# Autodesk Inventor assembly: Schlitten
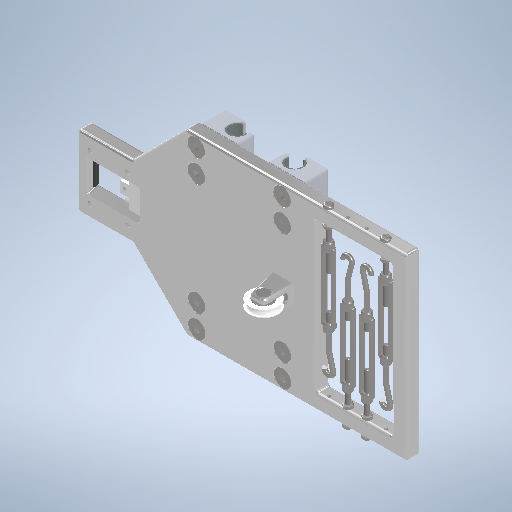
[picture p0: Inventor's stored thumbnail of the model, 512x512]
Saved by Autodesk Inventor 2025 (Build 290162010, 162A)
## iProperties
Created: 2024-11-25
Part Number: Schlitten
Document SubType Name: Assembly
Designer: Admin
Mass: 1140.3 g
Surface Area: 1828.97 cm^2
Volume: 452.563 cm^3
Density: 2.51965 g/cm^3
Author: Admin
## Documents named in this file (25)
- C:\Users\Admin\GIT\HDVKBM\CAD\Krandemonstrator\Schlitten.iam
- C:\Users\Admin\Documents\Inventor\Content Center Files\R2025\de-DE\BS 1804\BS 1804-2 - 2 x 10.ipt
- C:\Users\Admin\GIT\HDVKBM\CAD\Krandemonstrator\SchlittenS.ipt
- C:\Users\Admin\GIT\HDVKBM\CAD\Krandemonstrator\WJ200UM_01_10_1\WJ200UM_01_10_1.iam
- C:\Users\Admin\Documents\Inventor\Content Center Files\R2025\de-DE\DIN 7991(2)\DIN 7991 - M6x16.ipt
- C:\Users\Admin\Documents\Inventor\Content Center Files\R2025\de-DE\AS 1427(03)\AS 1427 - M2 x 10(1).ipt
- C:\Users\Admin\GIT\HDVKBM\CAD\Krandemonstrator\UmlenkrolleHalterHeavy.iam
- C:\Users\Admin\Documents\Inventor\Content Center Files\R2025\de-DE\DIN 7991(2)\DIN 7991 - M3x10.ipt
- C:\Users\Admin\GIT\HDVKBM\CAD\Krandemonstrator\Bremsbelag.ipt
- C:\Users\Admin\GIT\HDVKBM\CAD\Krandemonstrator\BremsePress.ipt
- C:\Users\Admin\GIT\HDVKBM\CAD\Krandemonstrator\Sliderhalterpress.ipt
- C:\Users\Admin\GIT\HDVKBM\CAD\Krandemonstrator\SchubstangeAPress.ipt
- C:\Users\Admin\GIT\HDVKBM\CAD\Krandemonstrator\SchubstangeAPressB.ipt
- C:\Users\Admin\GIT\HDVKBM\CAD\Krandemonstrator\SliderhalterpressB.ipt
- C:\Users\Admin\GIT\HDVKBM\CAD\Krandemonstrator\Druckfeder15.ipt
- C:\Users\Admin\GIT\HDVKBM\CAD\Krandemonstrator\Druckfeder16.ipt
- C:\Users\Admin\Documents\Inventor\Content Center Files\R2025\de-DE\DIN 934\DIN 934 - M3 x 0,5.ipt
- C:\Users\Admin\Documents\Inventor\Content Center Files\R2025\de-DE\AS 1427(01)\AS 1427 - M3 x 40(3).ipt
- C:\Users\Admin\GIT\HDVKBM\CAD\Krandemonstrator\Spannschloss M3-wie din1480.ipt
- C:\Users\Admin\GIT\HDVKBM\CAD\Krandemonstrator\M3 Haken 40mm.ipt
- C:\Users\Admin\Documents\Inventor\Content Center Files\R2025\de-DE\BS EN 28 740\ISO 8740 - 2 x 30(1).ipt
- C:\Users\Admin\GIT\HDVKBM\CAD\Krandemonstrator\Zugfeder16.ipt
- C:\Users\Admin\GIT\HDVKBM\CAD\PrintB\BremsbelagBreit.ipt
- C:\Users\Admin\GIT\HDVKBM\CAD\PrintB\Bauteil8.ipt
- C:\Users\Admin\Documents\Inventor\Content Center Files\R2025\de-DE\AS 1427(01)\AS 1427 - M3 x 35(3).ipt
## Components (57 placed, 23 different names)
1. SchlittenS:1 — Passend:1, Passend:2, Passend:3, Passend:4, Starr:17, Starr:15, Starr:18, Starr:16, Starr:2, Starr:3, Planar:6, Drehbar:9, Zylindrisch:33, Zylindrisch:35, Planar:8, Zylindrisch:39, Passend:40, Passend:41, Passend:42, Passend:43, Zylindrisch:40, Zylindrisch:41, Planar:10, Zylindrisch:50, Zylindrisch:51, Zylindrisch:52, Starr:34, Starr:35, Starr:36, Starr:37, Starr:38, Starr:39, Passend:50, Passend:52, Passend:54, Passend:56, Starr:48, Verschiebbar:34, Verschiebbar:32
2. DIN 7991 M3x10:6 — Zylindrisch:41
3. DIN 7991 M3x10:5 — Zylindrisch:40
4. DIN 934 - ersetzt durch DIN EN 24032/28673/28674 M3:2 — Passend:49, Passend:50
5. DIN 934 - ersetzt durch DIN EN 24032/28673/28674 M3:3 — Passend:51, Passend:52
6. DIN 934 - ersetzt durch DIN EN 24032/28673/28674 M3:4 — Passend:53, Passend:54
7. DIN 934 - ersetzt durch DIN EN 24032/28673/28674 M3:5 — Passend:55, Passend:56
8. AS 1427 - Metrisch M3 x 40:4 — Starr:36, Passend:53, Starr:40
9. AS 1427 - Metrisch M3 x 40:1 — Starr:38, Passend:51, Starr:43
10. AS 1427 - Metrisch M3 x 40:2 — Starr:39, Passend:49, Starr:42
11. AS 1427 - Metrisch M3 x 40:3 — Starr:37, Passend:55, Starr:41
12. Spannschloss M3-wie din1480:1 — Starr:40, Starr:45
13. Spannschloss M3-wie din1480:2 — Starr:41, Starr:44
14. Spannschloss M3-wie din1480:3 — Starr:42, Starr:47
15. Spannschloss M3-wie din1480:4 — Starr:43, Starr:46
16. M3 Haken 40mm:1 — Starr:44
17. M3 Haken 40mm:2 — Starr:45
18. M3 Haken 40mm:3 — Starr:46
19. M3 Haken 40mm:4 — Starr:47
20. UmlenkrolleHalterHeavy:1 [sub-assembly] — Planar:10
21. AS 1427 - Metrisch M3 x 35:1 — Starr:31, Passend:57, Passend:59, Passend:60
22. BremsePress:1 — Drehbar:9, Drehung:1, Starr:49, Kugelförmig:1
23. AS 1427 - Metrisch M2 x 10:20 — Passend:37, Zylindrisch:33, Drehung/Translation:1, Drehung:1
24. AS 1427 - Metrisch M2 x 10:21 — Passend:38, Zylindrisch:35
25. SchubstangeAPress:1 — Starr:31, Planar:13, Drehung/Translation:1, Passend:58, Verschiebbar:34
26. SchubstangeAPressB:1 — Verschiebbar:32, Starr:32, Starr:33
27. Druckfeder1:1 — Starr:33
28. Druckfeder1:1 — Starr:32, Planar:13
29. AS 1427 - Metrisch M2 x 10:22 — Passend:44, Zylindrisch:52
30. AS 1427 - Metrisch M2 x 10:23 — Passend:45, Zylindrisch:51
31. BS EN 28740 - ersetzt durch BS EN ISO 8740 2 x 30:1 — Starr:48, Drehbar:10, Zylindrisch:53
32. Zugfeder1:1 — Drehbar:10, Zylindrisch:53, Starr:51
33. BremsbelagBreit:1 — Starr:49
34. DIN 934 - ersetzt durch DIN EN 24032/28673/28674 M3:6 — Passend:57, Passend:58
35. DIN 934 - ersetzt durch DIN EN 24032/28673/28674 M3:7 — Passend:59, Passend:60
36. Sliderhalterpress:3 — Passend:37, Passend:38, Planar:8
37. AS 1427 - Metrisch M2 x 10:14 — Passend:31, Zylindrisch:39
38. AS 1427 - Metrisch M2 x 10:15 — Passend:32, Zylindrisch:50
39. SliderhalterpressB:1 — Passend:31, Passend:32, Planar:6, Passend:44, Passend:45
40. Bauteil8:2 — Verschiebbar:33, Kugelförmig:1
41. Bauteil8:1 — Starr:51, Verschiebbar:33
42. BS 1804 : Teil 2 2 x 10:7 — Starr:2
43. BS 1804 : Teil 2 2 x 10:8 — Starr:3
44. WJ200UM_01_10_1:1 [sub-assembly] — Starr:15
45. WJ200UM_01_10_1:2 [sub-assembly] — Starr:16
46. WJ200UM_01_10_1:3 [sub-assembly] — Starr:17
47. WJ200UM_01_10_1:4 [sub-assembly] — Starr:18
48. DIN 7991 M6x16:1 — Passend:1
49. DIN 7991 M6x16:2 — Passend:2
50. DIN 7991 M6x16:3 — Passend:3
51. DIN 7991 M6x16:5 — Passend:40
52. DIN 7991 M6x16:6 — Passend:41
53. DIN 7991 M6x16:7 — Passend:42
54. DIN 7991 M6x16:8 — Passend:43
55. DIN 7991 M6x16:4 — Passend:4
56. Bremsbelag:2 — Starr:34
57. Bremsbelag:1 — Starr:35
## Relationships (75: Mate 28, WeldJoint 26, CylindricalJoint 9, PlanarJoint 4, TranslationJoint 3, RevoluteJoint 2, RelateRotateTranslate 1, RelateRotation 1, BallJoint 1)
- Passend:1 [Mate]: SchlittenS:1 ↔ DIN 7991 M6x16:1
- Passend:2 [Mate]: SchlittenS:1 ↔ DIN 7991 M6x16:2
- Passend:3 [Mate]: SchlittenS:1 ↔ DIN 7991 M6x16:3
- Passend:4 [Mate]: SchlittenS:1 ↔ DIN 7991 M6x16:4
- Starr:17 [WeldJoint]: SchlittenS:1 ↔ WJ200UM_01_10_1:3
- Starr:15 [WeldJoint]: SchlittenS:1 ↔ WJ200UM_01_10_1:1
- Starr:18 [WeldJoint]: SchlittenS:1 ↔ WJ200UM_01_10_1:4
- Starr:16 [WeldJoint]: SchlittenS:1 ↔ WJ200UM_01_10_1:2
- Starr:2 [WeldJoint]: SchlittenS:1 ↔ BS 1804 : Teil 2 2 x 10:7
- Starr:3 [WeldJoint]: SchlittenS:1 ↔ BS 1804 : Teil 2 2 x 10:8
- [Mate]: DIN 7991 M3x10:5 ↔ UmlenkrolleHalterHeavy:1
- [Mate]: DIN 7991 M3x10:6 ↔ UmlenkrolleHalterHeavy:1
- Passend:31 [Mate]: AS 1427 - Metrisch M2 x 10:14 ↔ SliderhalterpressB:1
- Passend:32 [Mate]: AS 1427 - Metrisch M2 x 10:15 ↔ SliderhalterpressB:1
- Planar:6: SchlittenS:1 ↔ SliderhalterpressB:1
- Drehbar:9 [RevoluteJoint] (0.5 mm): SchlittenS:1 ↔ BremsePress:1
- Passend:37 [Mate]: AS 1427 - Metrisch M2 x 10:20 ↔ Sliderhalterpress:3
- Passend:38 [Mate]: AS 1427 - Metrisch M2 x 10:21 ↔ Sliderhalterpress:3
- Zylindrisch:33 [CylindricalJoint]: SchlittenS:1 ↔ AS 1427 - Metrisch M2 x 10:20
- Zylindrisch:35 [CylindricalJoint]: SchlittenS:1 ↔ AS 1427 - Metrisch M2 x 10:21
- Planar:8: SchlittenS:1 ↔ Sliderhalterpress:3
- Zylindrisch:39 [CylindricalJoint]: SchlittenS:1 ↔ AS 1427 - Metrisch M2 x 10:14
- Starr:31 [WeldJoint]: AS 1427 - Metrisch M3 x 35:1 ↔ SchubstangeAPress:1
- Verschiebbar:32 [TranslationJoint]: SchlittenS:1 ↔ SchubstangeAPressB:1
- Passend:40 [Mate]: SchlittenS:1 ↔ DIN 7991 M6x16:5
- Passend:41 [Mate]: SchlittenS:1 ↔ DIN 7991 M6x16:6
- Passend:42 [Mate]: SchlittenS:1 ↔ DIN 7991 M6x16:7
- Passend:43 [Mate]: SchlittenS:1 ↔ DIN 7991 M6x16:8
- Zylindrisch:40 [CylindricalJoint]: SchlittenS:1 ↔ DIN 7991 M3x10:5
- Zylindrisch:41 [CylindricalJoint]: SchlittenS:1 ↔ DIN 7991 M3x10:6
- Planar:10: SchlittenS:1 ↔ UmlenkrolleHalterHeavy:1
- Zylindrisch:50 [CylindricalJoint]: SchlittenS:1 ↔ AS 1427 - Metrisch M2 x 10:15
- Starr:32 [WeldJoint]: SchubstangeAPressB:1 ↔ Druckfeder1:1
- Starr:33 [WeldJoint]: SchubstangeAPressB:1 ↔ Druckfeder1:1
- Planar:13: SchubstangeAPress:1 ↔ Druckfeder1:1
- Passend:44 [Mate]: AS 1427 - Metrisch M2 x 10:22 ↔ SliderhalterpressB:1
- Passend:45 [Mate]: AS 1427 - Metrisch M2 x 10:23 ↔ SliderhalterpressB:1
- Zylindrisch:51 [CylindricalJoint]: SchlittenS:1 ↔ AS 1427 - Metrisch M2 x 10:23
- Zylindrisch:52 [CylindricalJoint]: SchlittenS:1 ↔ AS 1427 - Metrisch M2 x 10:22
- Starr:34 [WeldJoint]: SchlittenS:1 ↔ Bremsbelag:2
- Starr:35 [WeldJoint]: SchlittenS:1 ↔ Bremsbelag:1
- Starr:36 [WeldJoint]: SchlittenS:1 ↔ AS 1427 - Metrisch M3 x 40:4
- Starr:37 [WeldJoint]: SchlittenS:1 ↔ AS 1427 - Metrisch M3 x 40:3
- Starr:38 [WeldJoint]: SchlittenS:1 ↔ AS 1427 - Metrisch M3 x 40:1
- Starr:39 [WeldJoint]: SchlittenS:1 ↔ AS 1427 - Metrisch M3 x 40:2
- Passend:49 [Mate]: DIN 934 - ersetzt durch DIN EN 24032/28673/28674 M3:2 ↔ AS 1427 - Metrisch M3 x 40:2
- Passend:50 [Mate]: SchlittenS:1 ↔ DIN 934 - ersetzt durch DIN EN 24032/28673/28674 M3:2
- Passend:51 [Mate]: DIN 934 - ersetzt durch DIN EN 24032/28673/28674 M3:3 ↔ AS 1427 - Metrisch M3 x 40:1
- Passend:52 [Mate]: SchlittenS:1 ↔ DIN 934 - ersetzt durch DIN EN 24032/28673/28674 M3:3
- Passend:53 [Mate]: DIN 934 - ersetzt durch DIN EN 24032/28673/28674 M3:4 ↔ AS 1427 - Metrisch M3 x 40:4
- Passend:54 [Mate]: SchlittenS:1 ↔ DIN 934 - ersetzt durch DIN EN 24032/28673/28674 M3:4
- Passend:55 [Mate]: DIN 934 - ersetzt durch DIN EN 24032/28673/28674 M3:5 ↔ AS 1427 - Metrisch M3 x 40:3
- Passend:56 [Mate]: SchlittenS:1 ↔ DIN 934 - ersetzt durch DIN EN 24032/28673/28674 M3:5
- Starr:40 [WeldJoint]: AS 1427 - Metrisch M3 x 40:4 ↔ Spannschloss M3-wie din1480:1
- Starr:41 [WeldJoint]: AS 1427 - Metrisch M3 x 40:3 ↔ Spannschloss M3-wie din1480:2
- Starr:42 [WeldJoint]: AS 1427 - Metrisch M3 x 40:2 ↔ Spannschloss M3-wie din1480:3
- Starr:43 [WeldJoint]: AS 1427 - Metrisch M3 x 40:1 ↔ Spannschloss M3-wie din1480:4
- Starr:44 [WeldJoint]: Spannschloss M3-wie din1480:2 ↔ M3 Haken 40mm:1
- Starr:45 [WeldJoint]: Spannschloss M3-wie din1480:1 ↔ M3 Haken 40mm:2
- Starr:46 [WeldJoint]: Spannschloss M3-wie din1480:4 ↔ M3 Haken 40mm:3
- Starr:47 [WeldJoint]: Spannschloss M3-wie din1480:3 ↔ M3 Haken 40mm:4
- Drehung/Translation:1 [RelateRotateTranslate] (4500 mm): AS 1427 - Metrisch M2 x 10:20 ↔ SchubstangeAPress:1
- Drehung:1 [RelateRotation] (1 ul): BremsePress:1 ↔ AS 1427 - Metrisch M2 x 10:20
- Starr:48 [WeldJoint]: SchlittenS:1 ↔ BS EN 28740 - ersetzt durch BS EN ISO 8740 2 x 30:1
- Drehbar:10 [RevoluteJoint]: BS EN 28740 - ersetzt durch BS EN ISO 8740 2 x 30:1 ↔ Zugfeder1:1
- Starr:49 [WeldJoint]: BremsePress:1 ↔ BremsbelagBreit:1
- Passend:57 [Mate]: AS 1427 - Metrisch M3 x 35:1 ↔ DIN 934 - ersetzt durch DIN EN 24032/28673/28674 M3:6
- Passend:58 [Mate]: SchubstangeAPress:1 ↔ DIN 934 - ersetzt durch DIN EN 24032/28673/28674 M3:6
- Zylindrisch:53 [CylindricalJoint]: BS EN 28740 - ersetzt durch BS EN ISO 8740 2 x 30:1 ↔ Zugfeder1:1
- Starr:51 [WeldJoint]: Zugfeder1:1 ↔ Bauteil8:1
- Verschiebbar:33 [TranslationJoint] (0.7 mm): Bauteil8:2 ↔ Bauteil8:1
- Kugelförmig:1 [BallJoint]: BremsePress:1 ↔ Bauteil8:2
- Verschiebbar:34 [TranslationJoint]: SchlittenS:1 ↔ SchubstangeAPress:1
- Passend:59 [Mate]: AS 1427 - Metrisch M3 x 35:1 ↔ DIN 934 - ersetzt durch DIN EN 24032/28673/28674 M3:7
- Passend:60 [Mate]: AS 1427 - Metrisch M3 x 35:1 ↔ DIN 934 - ersetzt durch DIN EN 24032/28673/28674 M3:7
